# Autodesk Inventor assembly: Vertical Lift
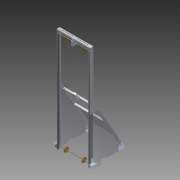
[picture p0: Inventor's stored thumbnail of the model, 180x180]
Saved by Autodesk Inventor 2015 (Build 190159000, 159)
## iProperties
Created: 2015-01-13
Part Number: Vertical Lift
Document SubType Name: Assembly
Designer: Jarod
Author: Jarod
## Documents named in this file (25)
- C:\Users\Jarod\Documents\Robotics\FRC\2015\CAD\Robot\Vertical Lift\Vertical Lift.iam
- C:\Users\Jarod\Documents\Robotics\FRC\2015\CAD\Robot\Vertical Lift\garage door 2in rail.ipt
- C:\Users\Jarod\Documents\Robotics\FRC\2015\CAD\Robot\Vertical Lift\rail aligner.ipt
- C:\Users\Jarod\Documents\Robotics\FRC\2015\CAD\Robot\Vertical Lift\garage door 2in rail_MIR.ipt
- C:\Users\Jarod\Documents\Robotics\FRC\2015\CAD\Robot\Vertical Lift\0.375 axle.ipt
- C:\Users\Jarod\Documents\Robotics\FRC\2015\CAD\Robot\Vertical Lift\Imported Components\0.375 shaft collar\0.375 shaft collar.ipt
- C:\Users\Jarod\Documents\Robotics\FRC\2015\CAD\Robot\Vertical Lift\Imported Components\Versaframe 60deg gusset\Versaframe 60deg gusset.ipt
- C:\Users\Jarod\Documents\Robotics\FRC\2015\CAD\Robot\Vertical Lift\1x1 support.ipt
- C:\Users\Jarod\Documents\Robotics\FRC\2015\CAD\Robot\Vertical Lift\garage door 3in pulley.ipt
- C:\Users\Jarod\Documents\Robotics\FRC\2015\CAD\Robot\Vertical Lift\1x1 horizontal support.ipt
- C:\Users\Jarod\Documents\Robotics\FRC\2015\CAD\Robot\Vertical Lift\camera mount.ipt
- C:\Users\Jarod\Documents\Robotics\FRC\2015\CAD\Robot\Vertical Lift\Imported Components\AXIS-M1011\AXIS-M1011.ipt
- C:\Users\Jarod\Documents\Robotics\FRC\2015\CAD\Robot\Vertical Lift\polycarb sheet.ipt
- C:\Users\Jarod\Documents\Robotics\FRC\2015\CAD\Robot\Vertical Lift\side panel.ipt
- C:\Users\Jarod\Documents\Robotics\FRC\2015\CAD\Robot\Vertical Lift\steel cable support.ipt
- C:\Users\Jarod\Documents\Robotics\FRC\2015\CAD\Robot\Vertical Lift\rail support 2x2 angle.ipt
- C:\Users\Jarod\Documents\Robotics\FRC\2015\CAD\Robot\Vertical Lift\rail support 2x1.ipt
- C:\Users\Jarod\Documents\Robotics\FRC\2015\CAD\Robot\Vertical Lift\rail support 2x2 angle_MIR.ipt
- C:\Users\Jarod\Documents\Robotics\FRC\2015\CAD\Robot\Vertical Lift\axle support 2x1.ipt
- C:\Users\Jarod\Documents\Robotics\FRC\2015\CAD\Robot\Vertical Lift\1x1 mechanical stop.ipt
- C:\Users\Jarod\Documents\Robotics\FRC\2015\CAD\Robot\Vertical Lift\mechanical stop 2x2 angle.ipt
- C:\Users\Jarod\Documents\Robotics\FRC\2015\CAD\Robot\Vertical Lift\mechanical stop 2x2 angle_MIR.ipt
- C:\Users\Jarod\Documents\Robotics\FRC\2015\CAD\Robot\Vertical Lift\mounting bracket.ipt
- C:\Users\Jarod\Documents\Robotics\FRC\2015\CAD\Robot\Vertical Lift\30deg gusset plate.ipt
- C:\Users\Jarod\Documents\Robotics\FRC\2015\CAD\Robot\Vertical Lift\wood gusset.ipt
## Components (58 placed, 24 different names)
1. garage door 2in rail:1 — Mate:44, Flush:5, Mate:45, Flush:7, Mate:48, Mate:108, Flush:24, Flush:26, Flush:64, Mate:296, Mate:297, Mate:298, Flush:80, Flush:81, Mate:332, Mate:334, Flush:82, Mate:335, Mate:336, Flush:84
2. garage door 2in rail_MIR:1 — Mate:46, Mate:47, Flush:6, Flush:7, Mate:48, Mate:98, Mate:106, Flush:24, Flush:25, Flush:65, Mate:300, Mate:303, Mate:304, Mate:337, Flush:83, Mate:338
3. mounting bracket:1 — Mate:334, Flush:82, Mate:335, Mate:336
4. mounting bracket:2 — Mate:337, Flush:83, Mate:338
5. rail aligner:1 — Mate:46, Mate:47, Flush:6
6. rail aligner:2 — Mate:44, Flush:5, Mate:45
7. 0.375 axle:1 — Mate:99, Mate:101, Mate:132, Mate:133, Mate:136, Mate:137, Mate:138, Mate:139, Mate:322, Mate:325
8. 0.375 axle:2 — Mate:98, Mate:103, Mate:105, Mate:107, Mate:109, Mate:134, Mate:135, Mate:144, Mate:145, Mate:146, Mate:147, Flush:74
9. garage door 3in pulley:1 — Mate:132, Mate:142, Mate:143, Flush:26, Flush:78
10. garage door 3in pulley:2 — Mate:133, Mate:140, Mate:141, Flush:25, Flush:79
11. garage door 3in pulley:3 — Mate:134, Mate:150, Mate:151, Flush:78
12. garage door 3in pulley:4 — Mate:135, Mate:148, Mate:149, Flush:79
13. 0.375 shaft collar:1 — Mate:99
14. 0.375 shaft collar:2 — Mate:101
15. 0.375 shaft collar:3 — Mate:103, Mate:300
16. 0.375 shaft collar:4 — Mate:105, Mate:106
17. 0.375 shaft collar:5 — Mate:107, Mate:108
18. 0.375 shaft collar:6 — Mate:109, Mate:299
19. 0.375 shaft collar:7 — Mate:136, Mate:140
20. 0.375 shaft collar:8 — Mate:137, Mate:141
21. 0.375 shaft collar:9 — Mate:138, Mate:142
22. 0.375 shaft collar:10 — Mate:139, Mate:143
23. 0.375 shaft collar:11 — Mate:144, Mate:148
24. 0.375 shaft collar:12 — Mate:145, Mate:149
25. 0.375 shaft collar:13 — Mate:146, Mate:150
26. 0.375 shaft collar:14 — Mate:147, Mate:151
27. Versaframe 60deg gusset:1 — Mate:117, Flush:81, Mate:346
28. Versaframe 60deg gusset:2 — Mate:293, Flush:66, Mate:347, Flush:92
29. Versaframe 60deg gusset:3 — Mate:119, Flush:16, Flush:69, Flush:92
30. Versaframe 60deg gusset:4 — Mate:294, Flush:68, Flush:69, Mate:340
31. 1x1 support:1 — Mate:117, Mate:275, Flush:60, Mate:290, Flush:62, Mate:293, Flush:66, Flush:90, Flush:91, Mate:343, Mate:346, Mate:347, Mate:349, Mate:350, Mate:352, Mate:355, Mate:357, Mate:363, Mate:364, Mate:366, Mate:367, Mate:377, Mate:378, Mate:379, Mate:380, Mate:383
32. 1x1 support:2 — Mate:119, Flush:16, Mate:276, Flush:63, Mate:291, Mate:294, Flush:68, Mate:340, Mate:348, Mate:351, Mate:353, Mate:356, Mate:358, Mate:369, Mate:370, Mate:372, Mate:373, Mate:375, Mate:376, Mate:381, Mate:382
33. 1x1 horizontal support:1 — Flush:91, Mate:343, Mate:348, Mate:365, Mate:374, Mate:387, Mate:388, Mate:389
34. 1x1 horizontal support:2 — Flush:90, Mate:349, Mate:368, Mate:371
35. camera mount:1 — Mate:384, Mate:385, Mate:386, Mate:387, Mate:388, Mate:389
36. AXIS-M1011:1 — Mate:384, Mate:385, Mate:386
37. rail support 2x2 angle:1 — Mate:296, Mate:297, Mate:298, Mate:299, Mate:301, Flush:71, Mate:302, Mate:318, Flush:77, Mate:341, Flush:85, Flush:86, Mate:344, Mate:361
38. rail support 2x2 angle_MIR:1 — Mate:303, Mate:304, Flush:72, Flush:74, Mate:320, Flush:87, Mate:342, Flush:88, Mate:345, Mate:360
39. 30deg gusset plate:1 — Mate:341, Flush:85, Flush:86
40. 30deg gusset plate:2 — Flush:87, Mate:342, Flush:88
41. wood gusset:1 — Mate:350, Mate:363, Mate:364, Mate:365
42. wood gusset:2 — Mate:351, Mate:372, Mate:373, Mate:374
43. wood gusset:3 — Mate:352, Mate:377, Mate:378
44. wood gusset:4 — Mate:353, Mate:375, Mate:376
45. wood gusset:5 — Mate:355, Mate:366, Mate:367, Mate:368
46. wood gusset:6 — Mate:356, Mate:369, Mate:370, Mate:371
47. wood gusset:7 — Mate:357, Mate:379, Mate:380
48. wood gusset:8 — Mate:358, Mate:381, Mate:382
49. rail support 2x1:1 — Mate:301, Flush:71, Mate:302, Flush:72, Mate:305, Flush:73
50. axle support 2x1:1 — Mate:305, Flush:73, Mate:316, Flush:75, Flush:76, Flush:77
51. 1x1 mechanical stop:1 — Mate:316, Flush:75, Flush:76
52. steel cable support:1 — Mate:318, Mate:344, Mate:360
53. steel cable support:2 — Mate:320, Mate:345, Mate:361
54. mechanical stop 2x2 angle:1 — Mate:322
55. mechanical stop 2x2 angle_MIR:1 — Mate:325
56. polycarb sheet:1 — Mate:275, Mate:276, Flush:60, Mate:383
57. side panel:1 — Mate:290, Flush:62, Flush:64, Flush:80, Mate:332, Flush:84
58. side panel:2 — Flush:63, Mate:291, Flush:65
## Relationships (146: Mate 110, Flush 36)
- Mate:44: garage door 2in rail:1 ↔ rail aligner:2
- Flush:5: garage door 2in rail:1 ↔ rail aligner:2
- Mate:45: garage door 2in rail:1 ↔ rail aligner:2
- Mate:46: garage door 2in rail_MIR:1 ↔ rail aligner:1
- Mate:47: garage door 2in rail_MIR:1 ↔ rail aligner:1
- Flush:6: garage door 2in rail_MIR:1 ↔ rail aligner:1
- Flush:7: garage door 2in rail:1 ↔ garage door 2in rail_MIR:1
- Mate:48 (-552.45 mm): garage door 2in rail:1 ↔ garage door 2in rail_MIR:1
- Mate:98: garage door 2in rail_MIR:1 ↔ 0.375 axle:2
- Mate:99: 0.375 axle:1 ↔ 0.375 shaft collar:1
- Mate:101: 0.375 axle:1 ↔ 0.375 shaft collar:2
- Mate:103: 0.375 axle:2 ↔ 0.375 shaft collar:3
- Mate:105: 0.375 axle:2 ↔ 0.375 shaft collar:4
- Mate:106: garage door 2in rail_MIR:1 ↔ 0.375 shaft collar:4
- Mate:107: 0.375 axle:2 ↔ 0.375 shaft collar:5
- Mate:108: garage door 2in rail:1 ↔ 0.375 shaft collar:5
- Mate:109: 0.375 axle:2 ↔ 0.375 shaft collar:6
- Mate:117: Versaframe 60deg gusset:1 ↔ 1x1 support:1
- Mate:119: Versaframe 60deg gusset:3 ↔ 1x1 support:2
- Flush:16: Versaframe 60deg gusset:3 ↔ 1x1 support:2
- Mate:132: 0.375 axle:1 ↔ garage door 3in pulley:1
- Mate:133: 0.375 axle:1 ↔ garage door 3in pulley:2
- Flush:24: garage door 2in rail:1 ↔ garage door 2in rail_MIR:1
- Mate:134: 0.375 axle:2 ↔ garage door 3in pulley:3
- Mate:135: 0.375 axle:2 ↔ garage door 3in pulley:4
- Mate:136: 0.375 axle:1 ↔ 0.375 shaft collar:7
- Mate:137: 0.375 axle:1 ↔ 0.375 shaft collar:8
- Mate:138: 0.375 axle:1 ↔ 0.375 shaft collar:9
- Mate:139: 0.375 axle:1 ↔ 0.375 shaft collar:10
- Mate:140: garage door 3in pulley:2 ↔ 0.375 shaft collar:7
- Mate:141: garage door 3in pulley:2 ↔ 0.375 shaft collar:8
- Mate:142: garage door 3in pulley:1 ↔ 0.375 shaft collar:9
- Mate:143: garage door 3in pulley:1 ↔ 0.375 shaft collar:10
- Mate:144: 0.375 axle:2 ↔ 0.375 shaft collar:11
- Mate:145: 0.375 axle:2 ↔ 0.375 shaft collar:12
- Mate:146: 0.375 axle:2 ↔ 0.375 shaft collar:13
- Mate:147: 0.375 axle:2 ↔ 0.375 shaft collar:14
- Mate:148: garage door 3in pulley:4 ↔ 0.375 shaft collar:11
- Mate:149: garage door 3in pulley:4 ↔ 0.375 shaft collar:12
- Mate:150: garage door 3in pulley:3 ↔ 0.375 shaft collar:13
- Mate:151: garage door 3in pulley:3 ↔ 0.375 shaft collar:14
- Flush:25 (-120.65 mm): garage door 2in rail_MIR:1 ↔ garage door 3in pulley:2
- Flush:26 (120.65 mm): garage door 2in rail:1 ↔ garage door 3in pulley:1
- Mate:275: 1x1 support:1 ↔ polycarb sheet:1
- Mate:276: 1x1 support:2 ↔ polycarb sheet:1
- Flush:60: 1x1 support:1 ↔ polycarb sheet:1
- Mate:290: 1x1 support:1 ↔ side panel:1
- Flush:62: 1x1 support:1 ↔ side panel:1
- Flush:63: 1x1 support:2 ↔ side panel:2
- Mate:291: 1x1 support:2 ↔ side panel:2
- Flush:64: garage door 2in rail:1 ↔ side panel:1
- Flush:65: garage door 2in rail_MIR:1 ↔ side panel:2
- Mate:293: Versaframe 60deg gusset:2 ↔ 1x1 support:1
- Flush:66: Versaframe 60deg gusset:2 ↔ 1x1 support:1
- Mate:294: Versaframe 60deg gusset:4 ↔ 1x1 support:2
- Flush:68: Versaframe 60deg gusset:4 ↔ 1x1 support:2
- Flush:69: Versaframe 60deg gusset:3 ↔ Versaframe 60deg gusset:4
- Mate:296: garage door 2in rail:1 ↔ rail support 2x2 angle:1
- Mate:297 (1.5875 mm): garage door 2in rail:1 ↔ rail support 2x2 angle:1
- Mate:298: garage door 2in rail:1 ↔ rail support 2x2 angle:1
- Mate:299: 0.375 shaft collar:6 ↔ rail support 2x2 angle:1
- Mate:300: garage door 2in rail_MIR:1 ↔ 0.375 shaft collar:3
- Mate:301: rail support 2x2 angle:1 ↔ rail support 2x1:1
- Flush:71: rail support 2x2 angle:1 ↔ rail support 2x1:1
- Mate:302: rail support 2x2 angle:1 ↔ rail support 2x1:1
- Mate:303: garage door 2in rail_MIR:1 ↔ rail support 2x2 angle_MIR:1
- Mate:304: garage door 2in rail_MIR:1 ↔ rail support 2x2 angle_MIR:1
- Flush:72: rail support 2x2 angle_MIR:1 ↔ rail support 2x1:1
- Mate:305: rail support 2x1:1 ↔ axle support 2x1:1
- Flush:73: rail support 2x1:1 ↔ axle support 2x1:1
- Flush:74 (-12.7 mm): 0.375 axle:2 ↔ rail support 2x2 angle_MIR:1
- Mate:316: axle support 2x1:1 ↔ 1x1 mechanical stop:1
- Flush:75: axle support 2x1:1 ↔ 1x1 mechanical stop:1
- Flush:76: axle support 2x1:1 ↔ 1x1 mechanical stop:1
- Mate:318: rail support 2x2 angle:1 ↔ steel cable support:1
- Mate:320: rail support 2x2 angle_MIR:1 ↔ steel cable support:2
- Mate:322: 0.375 axle:1 ↔ mechanical stop 2x2 angle:1
- Mate:325: 0.375 axle:1 ↔ mechanical stop 2x2 angle_MIR:1
- Flush:77 (-266.7 mm): rail support 2x2 angle:1 ↔ axle support 2x1:1
- Flush:78: garage door 3in pulley:1 ↔ garage door 3in pulley:3
- Flush:79: garage door 3in pulley:2 ↔ garage door 3in pulley:4
- Flush:80: garage door 2in rail:1 ↔ side panel:1
- Flush:81: garage door 2in rail:1 ↔ Versaframe 60deg gusset:1
- Mate:332: garage door 2in rail:1 ↔ side panel:1
- Mate:334: garage door 2in rail:1 ↔ mounting bracket:1
- Flush:82 (-38.1 mm): garage door 2in rail:1 ↔ mounting bracket:1
- Mate:335: garage door 2in rail:1 ↔ mounting bracket:1
- Mate:336: garage door 2in rail:1 ↔ mounting bracket:1
- Mate:337: garage door 2in rail_MIR:1 ↔ mounting bracket:2
- Flush:83 (-38.1 mm): garage door 2in rail_MIR:1 ↔ mounting bracket:2
- Mate:338: garage door 2in rail_MIR:1 ↔ mounting bracket:2
- Mate:340: Versaframe 60deg gusset:4 ↔ 1x1 support:2
- Flush:84: garage door 2in rail:1 ↔ side panel:1
- Mate:341: rail support 2x2 angle:1 ↔ 30deg gusset plate:1
- Flush:85: rail support 2x2 angle:1 ↔ 30deg gusset plate:1
- Flush:86: rail support 2x2 angle:1 ↔ 30deg gusset plate:1
- Flush:87: rail support 2x2 angle_MIR:1 ↔ 30deg gusset plate:2
- Mate:342: rail support 2x2 angle_MIR:1 ↔ 30deg gusset plate:2
- Flush:88: rail support 2x2 angle_MIR:1 ↔ 30deg gusset plate:2
- Flush:90: 1x1 support:1 ↔ 1x1 horizontal support:2
- Flush:91: 1x1 support:1 ↔ 1x1 horizontal support:1
- Mate:343: 1x1 support:1 ↔ 1x1 horizontal support:1
- Mate:344: rail support 2x2 angle:1 ↔ steel cable support:1
- Mate:345: rail support 2x2 angle_MIR:1 ↔ steel cable support:2
- Mate:346: Versaframe 60deg gusset:1 ↔ 1x1 support:1
- Mate:347: Versaframe 60deg gusset:2 ↔ 1x1 support:1
- Mate:348: 1x1 support:2 ↔ 1x1 horizontal support:1
- Mate:349: 1x1 support:1 ↔ 1x1 horizontal support:2
- Flush:92: Versaframe 60deg gusset:2 ↔ Versaframe 60deg gusset:3
- Mate:350: 1x1 support:1 ↔ wood gusset:1
- Mate:351: 1x1 support:2 ↔ wood gusset:2
- Mate:352: 1x1 support:1 ↔ wood gusset:3
- Mate:353: 1x1 support:2 ↔ wood gusset:4
- Mate:355: 1x1 support:1 ↔ wood gusset:5
- Mate:356: 1x1 support:2 ↔ wood gusset:6
- Mate:357: 1x1 support:1 ↔ wood gusset:7
- Mate:358: 1x1 support:2 ↔ wood gusset:8
- Mate:360: rail support 2x2 angle_MIR:1 ↔ steel cable support:1
- Mate:361: rail support 2x2 angle:1 ↔ steel cable support:2
- Mate:363: 1x1 support:1 ↔ wood gusset:1
- Mate:364: 1x1 support:1 ↔ wood gusset:1
- Mate:365: 1x1 horizontal support:1 ↔ wood gusset:1
- Mate:366: 1x1 support:1 ↔ wood gusset:5
- Mate:367: 1x1 support:1 ↔ wood gusset:5
- Mate:368: 1x1 horizontal support:2 ↔ wood gusset:5
- Mate:369: 1x1 support:2 ↔ wood gusset:6
- Mate:370: 1x1 support:2 ↔ wood gusset:6
- Mate:371: 1x1 horizontal support:2 ↔ wood gusset:6
- Mate:372: 1x1 support:2 ↔ wood gusset:2
- Mate:373: 1x1 support:2 ↔ wood gusset:2
- Mate:374: 1x1 horizontal support:1 ↔ wood gusset:2
- Mate:375: 1x1 support:2 ↔ wood gusset:4
- Mate:376: 1x1 support:2 ↔ wood gusset:4
- Mate:377: 1x1 support:1 ↔ wood gusset:3
- Mate:378: 1x1 support:1 ↔ wood gusset:3
- Mate:379: 1x1 support:1 ↔ wood gusset:7
- Mate:380: 1x1 support:1 ↔ wood gusset:7
- Mate:381: 1x1 support:2 ↔ wood gusset:8
- Mate:382: 1x1 support:2 ↔ wood gusset:8
- Mate:383: 1x1 support:1 ↔ polycarb sheet:1
- Mate:384: camera mount:1 ↔ AXIS-M1011:1
- Mate:385: camera mount:1 ↔ AXIS-M1011:1
- Mate:386: camera mount:1 ↔ AXIS-M1011:1
- Mate:387: 1x1 horizontal support:1 ↔ camera mount:1
- Mate:388: 1x1 horizontal support:1 ↔ camera mount:1
- Mate:389: 1x1 horizontal support:1 ↔ camera mount:1
